# Autodesk Inventor assembly: Radial Engine Assembly_Jen
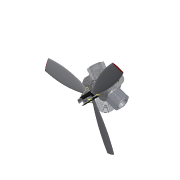
[picture p0: Inventor's stored thumbnail of the model, 180x180]
Saved by Autodesk Inventor 2022 Beta2 (Build 260130000, 130) ContinuousBuild 0
## iProperties
Created: 2013-03-12
Part Number: Radial Engine Assembly_Jen
Document SubType Name: Assembly
Designer: jmacmillan
Author: jmacmillan
## Documents named in this file (12)
- C:\Autodesk Inventor 2021 Intro Practice Files\Engine\Radial Engine Final2.iam
- C:\Autodesk Inventor 2021 Intro Practice Files\Engine\RBlock.ipt
- C:\Autodesk Inventor 2021 Intro Practice Files\Engine\Rcylinder.ipt
- C:\Autodesk Inventor 2021 Intro Practice Files\Engine\Crankshaft.ipt
- C:\Autodesk Inventor 2021 Intro Practice Files\Engine\Master Rod1.ipt
- C:\Autodesk Inventor 2021 Intro Practice Files\Engine\Piston head pin.ipt
- C:\Autodesk Inventor 2021 Intro Practice Files\Engine\Piston head.ipt
- C:\Autodesk Inventor 2021 Intro Practice Files\Engine\Hub.ipt
- C:\Autodesk Inventor 2021 Intro Practice Files\Engine\Shuttle.ipt
- C:\Autodesk Inventor 2021 Intro Practice Files\Engine\Pro_blade.ipt
- C:\Autodesk Inventor 2021 Intro Practice Files\Engine\Prop_Conrod.ipt
- C:\Autodesk Inventor 2021 Intro Practice Files\Engine\Connector Arm.ipt
## Components (30 placed, 11 different names)
1. RBlock:1 — Rigid:1, Cylindrical:2, Rigid:8, Rigid:9, Rigid:10, Rigid:11
2. Rcylinder:1 — Rigid:1, Cylindrical:1
3. Crankshaft:1 — Rotational:1, Cylindrical:2, Rigid:3
4. Master Rod1:1 — Rotational:1, Rotational:2, Cylindrical:22, Cylindrical:23, Cylindrical:21, Cylindrical:20
5. Piston head pin:1 — Rigid:2, Rotational:2
6. Piston head:1 — Rigid:2, Cylindrical:1
7. Hub:1 — Rigid:3, Cylindrical:3, Angle:1, Rotational:3, Rotational:4, Rotational:5
8. Shuttle:1 — Cylindrical:3, Angle:1, Ball:2, Ball:5, Ball:6
9. Pro_blade:1 — Rotational:3, Ball:1
10. Prop_Conrod:1 — Ball:1, Ball:2
11. Pro_blade:2 — Rotational:4
12. Prop_Conrod:2 — Ball:5
13. Pro_blade:3 — Rotational:5
14. Prop_Conrod:3 — Ball:6
15. Rcylinder:2 — Rigid:9
16. Piston head pin:2 — Rotational:6
17. Piston head:2
18. Rcylinder:3 — Rigid:10
19. Piston head pin:3 — Rotational:18
20. Piston head:3
21. Rcylinder:4 — Rigid:11
22. Piston head pin:4 — Rotational:14
23. Piston head:4
24. Rcylinder:5 — Rigid:8
25. Piston head pin:5 — Rotational:16
26. Piston head:5
27. Connector Arm:1 — Rotational:6, Cylindrical:22
28. Connector Arm:2 — Rotational:16, Cylindrical:21
29. Connector Arm:3 — Rotational:18, Cylindrical:20
30. Connector Arm:4 — Rotational:14, Cylindrical:23
## Relationships (38: WeldJoint 11, CylindricalJoint 11, RevoluteJoint 9, BallJoint 6, Angle 1)
- Rigid:1 [WeldJoint]: RBlock:1 ↔ Rcylinder:1
- Rotational:1 [RevoluteJoint] (-27.94 mm): Crankshaft:1 ↔ Master Rod1:1
- Rigid:2 [WeldJoint] (-1.27 mm): Piston head pin:1 ↔ Piston head:1
- Rotational:2 [RevoluteJoint]: Master Rod1:1 ↔ Piston head pin:1
- Cylindrical:1: Rcylinder:1 ↔ Piston head:1
- Cylindrical:2: RBlock:1 ↔ Crankshaft:1
- Rigid:3 [WeldJoint]: Crankshaft:1 ↔ Hub:1
- Cylindrical:3: Hub:1 ↔ Shuttle:1
- Angle:1 (180 deg): Hub:1 ↔ Shuttle:1
- Rotational:3 [RevoluteJoint]: Hub:1 ↔ Pro_blade:1
- Ball:1: Pro_blade:1 ↔ Prop_Conrod:1
- Ball:2: Shuttle:1 ↔ Prop_Conrod:1
- [BallJoint]: Pro_blade:2 ↔ Prop_Conrod:2
- [BallJoint]: Pro_blade:3 ↔ Prop_Conrod:3
- Rotational:4 [RevoluteJoint]: Hub:1 ↔ Pro_blade:2
- Ball:5: Shuttle:1 ↔ Prop_Conrod:2
- Rotational:5 [RevoluteJoint]: Hub:1 ↔ Pro_blade:3
- Ball:6: Shuttle:1 ↔ Prop_Conrod:3
- [WeldJoint] (-1.27 mm): Piston head pin:2 ↔ Piston head:2
- [CylindricalJoint]: Rcylinder:2 ↔ Piston head:2
- [WeldJoint] (-1.27 mm): Piston head pin:3 ↔ Piston head:3
- [CylindricalJoint]: Rcylinder:3 ↔ Piston head:3
- [WeldJoint] (-1.27 mm): Piston head pin:4 ↔ Piston head:4
- [CylindricalJoint]: Rcylinder:4 ↔ Piston head:4
- [WeldJoint] (-1.27 mm): Piston head pin:5 ↔ Piston head:5
- [CylindricalJoint]: Rcylinder:5 ↔ Piston head:5
- Rigid:8 [WeldJoint]: RBlock:1 ↔ Rcylinder:5
- Rigid:9 [WeldJoint]: RBlock:1 ↔ Rcylinder:2
- Rigid:10 [WeldJoint]: RBlock:1 ↔ Rcylinder:3
- Rigid:11 [WeldJoint]: RBlock:1 ↔ Rcylinder:4
- Rotational:6 [RevoluteJoint]: Piston head pin:2 ↔ Connector Arm:1
- Cylindrical:22: Master Rod1:1 ↔ Connector Arm:1
- Rotational:14 [RevoluteJoint]: Piston head pin:4 ↔ Connector Arm:4
- Cylindrical:23: Master Rod1:1 ↔ Connector Arm:4
- Rotational:16 [RevoluteJoint]: Piston head pin:5 ↔ Connector Arm:2
- Cylindrical:21: Master Rod1:1 ↔ Connector Arm:2
- Rotational:18 [RevoluteJoint]: Piston head pin:3 ↔ Connector Arm:3
- Cylindrical:20: Master Rod1:1 ↔ Connector Arm:3
## Named parameters: d32_d3 = -1.27 mm, d33_d6 = 90 deg, d34_d7 = 127.43534 mm, d35_d3 = -1.27 mm, d36_d6 = 90 deg, d37_d7 = 73.18838 mm, d38_d3 = -1.27 mm, d39_d6 = 180 deg, d40_d7 = 115.26806 mm, d41_d3 = -1.27 mm, d42_d6 = 90 deg, d43_d7 = 142.71613 mm
